# Autodesk Inventor assembly: Assembly1
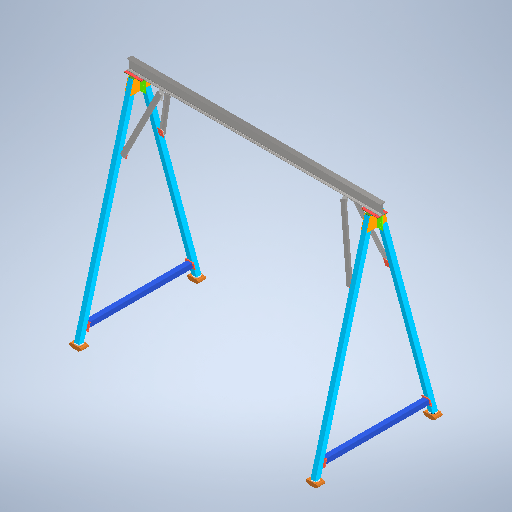
[picture p0: Inventor's stored thumbnail of the model, 512x512]
Saved by Autodesk Inventor 2025 (Build 290162010, 162A)
## iProperties
Created: 2024-06-11
Part Number: Assembly1
Document SubType Name: Assembly
Designer: admin
Stock Number: Кран козловой
Author: admin
## Documents named in this file (5)
- C:\Users\pokla\Documents\Inventor\Goat\ASY Goat.iam
- C:\Users\pokla\Documents\Inventor\Goat\WRS 000,000 кран козловой 6х4.ipt
- C:\Users\pokla\Documents\Inventor\Goat\Тельфер Таль электрическая.ipt
- C:\Users\pokla\Documents\Inventor\Goat\Support.iam
- C:\Users\pokla\Documents\Inventor\Goat\I-beam.ipt
## Components (5 placed, 4 different names)
1. WRS 000,000 кран козловой 6х4.ipt:1 — Mate:2, Mate:3, Flush:3
2. Тельфер Таль электрическая.ipt:1 — Mate:4
3. Support.iam:1 [sub-assembly] — Flush:24, Flush:25, Flush:26
4. Support.iam:2 [sub-assembly] — Flush:27, Mate:5, Mate:6
5. I-beam.ipt:1 — Mate:7, Flush:28
## Relationships (14: Flush 8, Mate 6)
- Mate:2: WRS 000,000 кран козловой 6х4.ipt:1
- Mate:3: WRS 000,000 кран козловой 6х4.ipt:1
- Flush:3: WRS 000,000 кран козловой 6х4.ipt:1
- Mate:4: Тельфер Таль электрическая.ipt:1
- [Flush]: Support.iam:1
- [Flush]: Support.iam:1
- Flush:24: Support.iam:1
- Flush:25: Support.iam:1
- Flush:26 (-2800 mm): Support.iam:1
- Flush:27: Support.iam:2
- Mate:5: Support.iam:2
- Mate:6 (-2800 mm): Support.iam:2
- Mate:7: I-beam.ipt:1
- Flush:28: I-beam.ipt:1
